# Autodesk Inventor assembly: CougSat-1
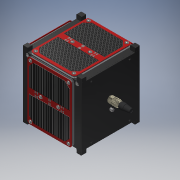
[picture p0: Inventor's stored thumbnail of the model, 180x180]
Saved by Autodesk Inventor 2018 (Build 220112000, 112)
## iProperties
Created: 2018-07-04
Part Number: CougSat-1
Document SubType Name: Assembly
Designer: Bradley
Author: Bradley
## Documents named in this file (5)
- D:\Users\Bradley\Documents\CougsInSpace\CougSat1-Hardware\CougSat1\CADModel\Native\CougSat-1.iam
- D:\Users\Bradley\Documents\CougsInSpace\CougSat1-Hardware\CougSat1-Structure\CADModel\Native\Structure.iam
- D:\Users\Bradley\Documents\CougsInSpace\CougSat1-Hardware\CougSat1-PowerBoard\CADModel\Native\EPS.iam
- D:\Users\Bradley\Documents\CougsInSpace\CougSat1-Hardware\CougSat1-PowerBoard\CADModel\Native\SolarPanel.iam
- D:\Users\Bradley\Documents\CougsInSpace\Resources\ComponentModels\Connectors\SODIMM-DDR.ipt
## Components (7 placed, 4 different names)
1. Structure:1 [sub-assembly] — Mate:1, Flush:2, Insert:1, Insert:2, Insert:3, Insert:4, Insert:5, Insert:6, Mate:9, Flush:7, Insert:7, Insert:8
2. EPS:1 [sub-assembly] — Flush:1, Mate:1, Flush:2
3. SolarPanel:1 [sub-assembly] — Insert:1, Insert:2
4. SolarPanel:2 [sub-assembly] — Insert:3, Insert:4
5. SolarPanel:3 [sub-assembly] — Insert:7, Insert:8
6. SolarPanel:4 [sub-assembly] — Insert:5, Insert:6
7. SODIMM-DDR:1 — Mate:9, Mate:8, Flush:7
## Relationships (14: Insert 8, Flush 3, Mate 3)
- Flush:1: EPS:1
- Mate:1 (0.04 mm): Structure:1 ↔ EPS:1
- Flush:2 (2 mm): Structure:1 ↔ EPS:1
- Insert:1: Structure:1 ↔ SolarPanel:1
- Insert:2: Structure:1 ↔ SolarPanel:1
- Insert:3: Structure:1 ↔ SolarPanel:2
- Insert:4: Structure:1 ↔ SolarPanel:2
- Insert:5: Structure:1 ↔ SolarPanel:4
- Insert:6: Structure:1 ↔ SolarPanel:4
- Mate:9 (0.55 mm): Structure:1 ↔ SODIMM-DDR:1
- Mate:8: SODIMM-DDR:1
- Flush:7 (-1.1 mm): Structure:1 ↔ SODIMM-DDR:1
- Insert:7: Structure:1 ↔ SolarPanel:3
- Insert:8: Structure:1 ↔ SolarPanel:3
